# Autodesk Inventor assembly: SinglePulley
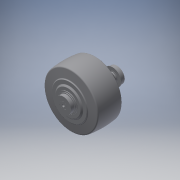
[picture p0: Inventor's stored thumbnail of the model, 180x180]
Saved by Autodesk Inventor 2016 (Build 200138000, 138)
## iProperties
Created: 2017-01-15
Part Number: SinglePulley
Document SubType Name: Assembly
Designer: Kyle
Author: Kyle
## Documents named in this file (6)
- F:\FRC\2017\DriveTrainRev2\Individual Parts\SinglePulley.iam
- F:\FRC\2017\DriveTrainRev2\Individual Parts\.5Bearing.ipt
- F:\FRC\2017\DriveTrainRev2\Individual Parts\3.875Churro.ipt
- F:\FRC\2017\DriveTrainRev2\Individual Parts\4x2Colson.ipt
- F:\FRC\2017\DriveTrainRev2\Individual Parts\24t9MMPulley6mm.ipt
- F:\FRC\2017\DriveTrainRev2\Individual Parts\.441Spacer.ipt
## Components (7 placed, 5 different names)
1. .5Bearing:1 — Mate:1, Flush:1, Mate:3
2. 3.875Churro:1 — Mate:1, Flush:1, Mate:2, Mate:14, Mate:15, Mate:18
3. 4x2Colson:1 — Mate:2, Mate:3, Mate:11
4. 24t9MMPulley6mm:1 — Mate:11, Mate:16, Mate:17
5. .5Bearing:2 — Mate:14, Mate:19
6. 24t9MMPulley6mm:2 — Mate:15, Mate:16, Mate:17
7. .441Spacer:1 — Mate:18, Mate:19
## Relationships (11: Mate 10, Flush 1)
- Mate:1: .5Bearing:1 ↔ 3.875Churro:1
- Flush:1: .5Bearing:1 ↔ 3.875Churro:1
- Mate:2: 3.875Churro:1 ↔ 4x2Colson:1
- Mate:3: .5Bearing:1 ↔ 4x2Colson:1
- Mate:11: 4x2Colson:1 ↔ 24t9MMPulley6mm:1
- Mate:14: 3.875Churro:1 ↔ .5Bearing:2
- Mate:15: 3.875Churro:1 ↔ 24t9MMPulley6mm:2
- Mate:16: 24t9MMPulley6mm:1 ↔ 24t9MMPulley6mm:2
- Mate:17: 24t9MMPulley6mm:1 ↔ 24t9MMPulley6mm:2
- Mate:18: 3.875Churro:1 ↔ .441Spacer:1
- Mate:19: .5Bearing:2 ↔ .441Spacer:1
